# Autodesk Inventor assembly: Turdbot Drivetrain
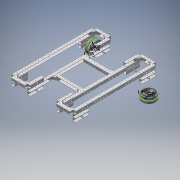
[picture p0: Inventor's stored thumbnail of the model, 180x180]
Saved by Autodesk Inventor 2016 (Build 200138000, 138)
## iProperties
Created: 2016-01-13
Part Number: Turdbot Drivetrain
Document SubType Name: Assembly
Designer: Administrator
Author: Administrator
## Documents named in this file (8)
- C:\Users\Administrator\Desktop\3192CAD\InitialRobotProto\Turdbot Drivetrain.iam
- C:\Users\Administrator\Desktop\3192CAD\InitialRobotProto\DBK_C-Channel_am-2222.ipt
- C:\Users\Administrator\Desktop\3192CAD\InitialRobotProto\DBK_CornerConnect_am-0212.ipt
- C:\Users\Administrator\Desktop\3192CAD\InitialRobotProto\WheelMountStack.iam
- C:\Users\Administrator\Desktop\3192CAD\InitialRobotProto\Wheelaxles.ipt
- C:\Users\Administrator\Desktop\3192CAD\InitialRobotProto\DBK_C-Channel_Tiny.ipt
- C:\Users\Administrator\Desktop\3192CAD\InitialRobotProto\DBK_C-Channel_tenlen.ipt
- C:\Users\Administrator\Desktop\3192CAD\InitialRobotProto\WheelPart.ipt
## Components (40 placed, 7 different names)
1. DBK_C-Channel_am-2222:1 — Mate:1, Mate:2, Mate:3, Mate:16, Mate:17, Mate:18, Mate:40, Mate:41, Mate:42, Mate:43, Mate:44, Mate:45
2. DBK_C-Channel_am-2222:4 — Mate:10, Mate:11, Mate:12, Mate:13, Mate:14, Mate:15, Mate:52, Mate:53, Mate:54, Mate:55, Mate:56, Mate:57
3. DBK_CornerConnect_am-0212:1 — Mate:10, Mate:11, Mate:12, Mate:106, Mate:107
4. DBK_CornerConnect_am-0212:2 — Mate:16, Mate:17, Mate:18, Mate:91, Mate:93
5. DBK_CornerConnect_am-0212:3 — Mate:1, Mate:2, Mate:3, Mate:94, Mate:96, Mate:98
6. DBK_CornerConnect_am-0212:4 — Mate:13, Mate:14, Mate:15, Mate:101, Mate:102
7. WheelMountStack:1 [sub-assembly] — Mate:55, Mate:56, Mate:57, Mate:60
8. WheelMountStack:2 [sub-assembly] — Mate:52, Mate:53, Mate:54, Mate:59
9. WheelMountStack:6 [sub-assembly] — Mate:43, Mate:44, Mate:45, Mate:144
10. WheelMountStack:7 [sub-assembly] — Mate:40, Mate:41, Mate:42
11. Wheelaxles:1 — Mate:143, Mate:144
12. Wheelaxles:2 — Mate:59
13. Wheelaxles:3 — Mate:60
14. Wheelaxles:4
15. DBK_C-Channel_am-2222:5 — Mate:85, Mate:86, Mate:87, Mate:109, Mate:110, Mate:111, Mate:112, Mate:114, Mate:124, Mate:125, Mate:126, Mate:127, Mate:128, Mate:129
16. DBK_C-Channel_Tiny:1 — Mate:73, Mate:74, Mate:75, Mate:88
17. DBK_C-Channel_Tiny:2 — Mate:82, Mate:83, Mate:84, Mate:85, Mate:87
18. DBK_C-Channel_Tiny:3 — Mate:76, Mate:77, Mate:78, Mate:89, Mate:90
19. DBK_C-Channel_Tiny:4 — Mate:79, Mate:80, Mate:81, Mate:86, Mate:113
20. DBK_CornerConnect_am-0212:5 — Mate:76, Mate:77, Mate:78, Mate:99, Mate:100, Mate:103
21. DBK_CornerConnect_am-0212:6 — Mate:82, Mate:83, Mate:84, Mate:95, Mate:97
22. DBK_CornerConnect_am-0212:7 — Mate:73, Mate:74, Mate:75, Mate:104, Mate:105, Mate:108
23. DBK_CornerConnect_am-0212:8 — Mate:79, Mate:80, Mate:81, Mate:92
24. DBK_CornerConnect_am-0212:9 — Mate:121, Mate:122, Mate:123, Mate:138, Mate:139
25. DBK_CornerConnect_am-0212:10 — Mate:124, Mate:125, Mate:126, Mate:140, Mate:141, Mate:142
26. DBK_CornerConnect_am-0212:11 — Mate:130, Mate:131, Mate:132, Mate:135, Mate:136, Mate:137
27. DBK_CornerConnect_am-0212:12 — Mate:127, Mate:128, Mate:129, Mate:133, Mate:134
28. DBK_C-Channel_am-2222:6 — Mate:88, Mate:89, Mate:90, Mate:115, Mate:116, Mate:117, Mate:118, Mate:119, Mate:120, Mate:121, Mate:122, Mate:123, Mate:130, Mate:131, Mate:132
29. DBK_C-Channel_Tiny:5 — Mate:94, Mate:95, Mate:96, Mate:97, Mate:98
30. DBK_C-Channel_Tiny:6 — Mate:104, Mate:105, Mate:106, Mate:107, Mate:108
31. DBK_C-Channel_Tiny:7 — Mate:99, Mate:100, Mate:101, Mate:102, Mate:103
32. DBK_C-Channel_Tiny:8 — Mate:91, Mate:92, Mate:93
33. DBK_C-Channel_Tiny:9 — Mate:118, Mate:119, Mate:120
34. DBK_C-Channel_Tiny:10 — Mate:115, Mate:116, Mate:117
35. DBK_C-Channel_Tiny:11 — Mate:109, Mate:110, Mate:111
36. DBK_C-Channel_Tiny:12 — Mate:112, Mate:113, Mate:114
37. DBK_C-Channel_tenlen:1 — Mate:133, Mate:134, Mate:135, Mate:136, Mate:137
38. DBK_C-Channel_tenlen:2 — Mate:138, Mate:139, Mate:140, Mate:141, Mate:142
39. WheelPart:1 — Mate:143
40. WheelPart:2
## Relationships (98: Mate 98)
- Mate:1: DBK_C-Channel_am-2222:1 ↔ DBK_CornerConnect_am-0212:3
- Mate:2: DBK_C-Channel_am-2222:1 ↔ DBK_CornerConnect_am-0212:3
- Mate:3: DBK_C-Channel_am-2222:1 ↔ DBK_CornerConnect_am-0212:3
- Mate:10: DBK_C-Channel_am-2222:4 ↔ DBK_CornerConnect_am-0212:1
- Mate:11: DBK_C-Channel_am-2222:4 ↔ DBK_CornerConnect_am-0212:1
- Mate:12: DBK_C-Channel_am-2222:4 ↔ DBK_CornerConnect_am-0212:1
- Mate:13: DBK_C-Channel_am-2222:4 ↔ DBK_CornerConnect_am-0212:4
- Mate:14: DBK_C-Channel_am-2222:4 ↔ DBK_CornerConnect_am-0212:4
- Mate:15: DBK_C-Channel_am-2222:4 ↔ DBK_CornerConnect_am-0212:4
- Mate:16: DBK_C-Channel_am-2222:1 ↔ DBK_CornerConnect_am-0212:2
- Mate:17: DBK_C-Channel_am-2222:1 ↔ DBK_CornerConnect_am-0212:2
- Mate:18: DBK_C-Channel_am-2222:1 ↔ DBK_CornerConnect_am-0212:2
- Mate:40: DBK_C-Channel_am-2222:1 ↔ WheelMountStack:7
- Mate:41: DBK_C-Channel_am-2222:1 ↔ WheelMountStack:7
- Mate:42: DBK_C-Channel_am-2222:1 ↔ WheelMountStack:7
- Mate:43: DBK_C-Channel_am-2222:1 ↔ WheelMountStack:6
- Mate:44: DBK_C-Channel_am-2222:1 ↔ WheelMountStack:6
- Mate:45: DBK_C-Channel_am-2222:1 ↔ WheelMountStack:6
- Mate:52: DBK_C-Channel_am-2222:4 ↔ WheelMountStack:2
- Mate:53: DBK_C-Channel_am-2222:4 ↔ WheelMountStack:2
- Mate:54: DBK_C-Channel_am-2222:4 ↔ WheelMountStack:2
- Mate:55: DBK_C-Channel_am-2222:4 ↔ WheelMountStack:1
- Mate:56: DBK_C-Channel_am-2222:4 ↔ WheelMountStack:1
- Mate:57: DBK_C-Channel_am-2222:4 ↔ WheelMountStack:1
- Mate:59: WheelMountStack:2 ↔ Wheelaxles:2
- Mate:60: WheelMountStack:1 ↔ Wheelaxles:3
- Mate:73: DBK_C-Channel_Tiny:1 ↔ DBK_CornerConnect_am-0212:7
- Mate:74: DBK_C-Channel_Tiny:1 ↔ DBK_CornerConnect_am-0212:7
- Mate:75: DBK_C-Channel_Tiny:1 ↔ DBK_CornerConnect_am-0212:7
- Mate:76: DBK_C-Channel_Tiny:3 ↔ DBK_CornerConnect_am-0212:5
- Mate:77: DBK_C-Channel_Tiny:3 ↔ DBK_CornerConnect_am-0212:5
- Mate:78: DBK_C-Channel_Tiny:3 ↔ DBK_CornerConnect_am-0212:5
- Mate:79: DBK_C-Channel_Tiny:4 ↔ DBK_CornerConnect_am-0212:8
- Mate:80: DBK_C-Channel_Tiny:4 ↔ DBK_CornerConnect_am-0212:8
- Mate:81: DBK_C-Channel_Tiny:4 ↔ DBK_CornerConnect_am-0212:8
- Mate:82: DBK_C-Channel_Tiny:2 ↔ DBK_CornerConnect_am-0212:6
- Mate:83: DBK_C-Channel_Tiny:2 ↔ DBK_CornerConnect_am-0212:6
- Mate:84: DBK_C-Channel_Tiny:2 ↔ DBK_CornerConnect_am-0212:6
- Mate:85: DBK_C-Channel_am-2222:5 ↔ DBK_C-Channel_Tiny:2
- Mate:86: DBK_C-Channel_am-2222:5 ↔ DBK_C-Channel_Tiny:4
- Mate:87: DBK_C-Channel_am-2222:5 ↔ DBK_C-Channel_Tiny:2
- Mate:88: DBK_C-Channel_Tiny:1 ↔ DBK_C-Channel_am-2222:6
- Mate:89: DBK_C-Channel_Tiny:3 ↔ DBK_C-Channel_am-2222:6
- Mate:90: DBK_C-Channel_Tiny:3 ↔ DBK_C-Channel_am-2222:6
- Mate:91: DBK_CornerConnect_am-0212:2 ↔ DBK_C-Channel_Tiny:8
- Mate:92: DBK_CornerConnect_am-0212:8 ↔ DBK_C-Channel_Tiny:8
- Mate:93: DBK_CornerConnect_am-0212:2 ↔ DBK_C-Channel_Tiny:8
- Mate:94: DBK_CornerConnect_am-0212:3 ↔ DBK_C-Channel_Tiny:5
- Mate:95: DBK_CornerConnect_am-0212:6 ↔ DBK_C-Channel_Tiny:5
- Mate:96: DBK_CornerConnect_am-0212:3 ↔ DBK_C-Channel_Tiny:5
- Mate:97: DBK_CornerConnect_am-0212:6 ↔ DBK_C-Channel_Tiny:5
- Mate:98: DBK_CornerConnect_am-0212:3 ↔ DBK_C-Channel_Tiny:5
- Mate:99: DBK_CornerConnect_am-0212:5 ↔ DBK_C-Channel_Tiny:7
- Mate:100: DBK_CornerConnect_am-0212:5 ↔ DBK_C-Channel_Tiny:7
- Mate:101: DBK_CornerConnect_am-0212:4 ↔ DBK_C-Channel_Tiny:7
- Mate:102: DBK_CornerConnect_am-0212:4 ↔ DBK_C-Channel_Tiny:7
- Mate:103: DBK_CornerConnect_am-0212:5 ↔ DBK_C-Channel_Tiny:7
- Mate:104: DBK_CornerConnect_am-0212:7 ↔ DBK_C-Channel_Tiny:6
- Mate:105: DBK_CornerConnect_am-0212:7 ↔ DBK_C-Channel_Tiny:6
- Mate:106: DBK_CornerConnect_am-0212:1 ↔ DBK_C-Channel_Tiny:6
- Mate:107: DBK_CornerConnect_am-0212:1 ↔ DBK_C-Channel_Tiny:6
- Mate:108: DBK_CornerConnect_am-0212:7 ↔ DBK_C-Channel_Tiny:6
- Mate:109: DBK_C-Channel_am-2222:5 ↔ DBK_C-Channel_Tiny:11
- Mate:110: DBK_C-Channel_am-2222:5 ↔ DBK_C-Channel_Tiny:11
- Mate:111: DBK_C-Channel_am-2222:5 ↔ DBK_C-Channel_Tiny:11
- Mate:112: DBK_C-Channel_am-2222:5 ↔ DBK_C-Channel_Tiny:12
- Mate:113: DBK_C-Channel_Tiny:4 ↔ DBK_C-Channel_Tiny:12
- Mate:114: DBK_C-Channel_am-2222:5 ↔ DBK_C-Channel_Tiny:12
- Mate:115: DBK_C-Channel_am-2222:6 ↔ DBK_C-Channel_Tiny:10
- Mate:116: DBK_C-Channel_am-2222:6 ↔ DBK_C-Channel_Tiny:10
- Mate:117: DBK_C-Channel_am-2222:6 ↔ DBK_C-Channel_Tiny:10
- Mate:118: DBK_C-Channel_am-2222:6 ↔ DBK_C-Channel_Tiny:9
- Mate:119: DBK_C-Channel_am-2222:6 ↔ DBK_C-Channel_Tiny:9
- Mate:120: DBK_C-Channel_am-2222:6 ↔ DBK_C-Channel_Tiny:9
- Mate:121: DBK_CornerConnect_am-0212:9 ↔ DBK_C-Channel_am-2222:6
- Mate:122: DBK_CornerConnect_am-0212:9 ↔ DBK_C-Channel_am-2222:6
- Mate:123: DBK_CornerConnect_am-0212:9 ↔ DBK_C-Channel_am-2222:6
- Mate:124: DBK_C-Channel_am-2222:5 ↔ DBK_CornerConnect_am-0212:10
- Mate:125: DBK_C-Channel_am-2222:5 ↔ DBK_CornerConnect_am-0212:10
- Mate:126: DBK_C-Channel_am-2222:5 ↔ DBK_CornerConnect_am-0212:10
- Mate:127: DBK_C-Channel_am-2222:5 ↔ DBK_CornerConnect_am-0212:12
- Mate:128: DBK_C-Channel_am-2222:5 ↔ DBK_CornerConnect_am-0212:12
- Mate:129: DBK_C-Channel_am-2222:5 ↔ DBK_CornerConnect_am-0212:12
- Mate:130: DBK_CornerConnect_am-0212:11 ↔ DBK_C-Channel_am-2222:6
- Mate:131: DBK_CornerConnect_am-0212:11 ↔ DBK_C-Channel_am-2222:6
- Mate:132: DBK_CornerConnect_am-0212:11 ↔ DBK_C-Channel_am-2222:6
- Mate:133: DBK_CornerConnect_am-0212:12 ↔ DBK_C-Channel_tenlen:1
- Mate:134: DBK_CornerConnect_am-0212:12 ↔ DBK_C-Channel_tenlen:1
- Mate:135: DBK_CornerConnect_am-0212:11 ↔ DBK_C-Channel_tenlen:1
- Mate:136: DBK_CornerConnect_am-0212:11 ↔ DBK_C-Channel_tenlen:1
- Mate:137: DBK_CornerConnect_am-0212:11 ↔ DBK_C-Channel_tenlen:1
- Mate:138: DBK_CornerConnect_am-0212:9 ↔ DBK_C-Channel_tenlen:2
- Mate:139: DBK_CornerConnect_am-0212:9 ↔ DBK_C-Channel_tenlen:2
- Mate:140: DBK_CornerConnect_am-0212:10 ↔ DBK_C-Channel_tenlen:2
- Mate:141: DBK_CornerConnect_am-0212:10 ↔ DBK_C-Channel_tenlen:2
- Mate:142: DBK_CornerConnect_am-0212:10 ↔ DBK_C-Channel_tenlen:2
- Mate:143: Wheelaxles:1 ↔ WheelPart:1
- Mate:144: WheelMountStack:6 ↔ Wheelaxles:1
